# Autodesk Inventor assembly: SolenoidValve
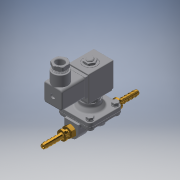
[picture p0: Inventor's stored thumbnail of the model, 180x180]
Saved by Autodesk Inventor 2018 (Build 220112000, 112)
## iProperties
Created: 2020-03-29
Part Number: SolenoidValve
Document SubType Name: Assembly
Designer: emile
Author: emile
## Documents named in this file (3)
- C:\Users\emile\OneDrive\Documents\GitHub\VentilatorCovid19\Respirator\MultiLine\SolenoidValve.iam
- C:\Users\emile\OneDrive\Documents\GitHub\VentilatorCovid19\Respirator\Peep\AirPressure\4711K513_BRASS SOLENOID VALVE.ipt
- C:\Users\emile\OneDrive\Documents\GitHub\VentilatorCovid19\Respirator\Peep\AirPressure\Brass Barbed Hose Fitting for Air and Water.ipt
## Components (3 placed, 2 different names)
1. 4711K513_BRASS SOLENOID VALVE:1
2. Brass Barbed Hose Fitting for Air and Water:1
3. Brass Barbed Hose Fitting for Air and Water:2
## Relationships (4: Mate 4)
- [Mate]: 4711K513_BRASS SOLENOID VALVE:1 ↔ Brass Barbed Hose Fitting for Air and Water:1
- [Mate]: 4711K513_BRASS SOLENOID VALVE:1 ↔ Brass Barbed Hose Fitting for Air and Water:2
- [Mate]: 4711K513_BRASS SOLENOID VALVE:1 ↔ Brass Barbed Hose Fitting for Air and Water:2
- [Mate]: 4711K513_BRASS SOLENOID VALVE:1 ↔ Brass Barbed Hose Fitting for Air and Water:1
